# Autodesk Inventor assembly: face
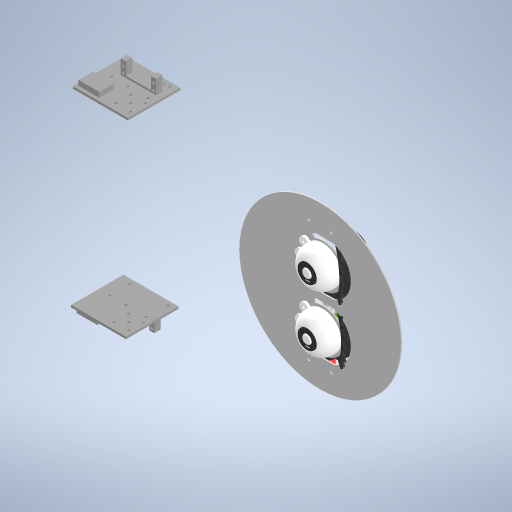
[picture p0: Inventor's stored thumbnail of the model, 512x512]
Saved by Autodesk Inventor 2023.2 (Build 272271030, 271C)
## iProperties
Created: 2024-01-26
Part Number: face
Document SubType Name: Assembly
Designer: I9232
Author: I9232
## Documents named in this file (5)
- D:\!project\fox_n_crow_construction\crow\face\face.iam
- D:\!project\fox_n_crow_construction\crow\face\Сборка глаза вороны.iam
- C:\Users\I9232\OneDrive\Рабочий стол\Проект\Модели\Ворона\Деталь1.ipt
- C:\Users\I9232\OneDrive\Рабочий стол\Платформа для крыльев лево\Платформа для крыльев лево.ipt
- C:\Users\I9232\OneDrive\Рабочий стол\Платформа для крыльев право\Платформа для крыльев право.ipt
## Components (4 placed, 4 different names)
1. Сборка глаза вороны:1 [sub-assembly] — Заподлицо:1
2. Деталь1:1 — Заподлицо:1
3. Платформа для крыльев лево:1
4. Платформа для крыльев право:1
## Relationships (1: Flush 1)
- Заподлицо:1 [Flush]: Сборка глаза вороны:1 ↔ Деталь1:1
